# Autodesk Inventor assembly: Assembly1
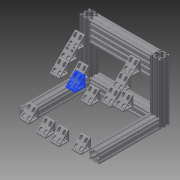
[picture p0: Inventor's stored thumbnail of the model, 180x180]
Saved by Autodesk Inventor 2014 (Build 180170000, 170)
## iProperties
Created: 2014-08-08
Part Number: Assembly1
Document SubType Name: Assembly
Designer: Matthew
Author: Matthew
## Documents named in this file (4)
- C:\Users\Matthew\Documents\GitHub\CNC Mill\Imported Components\8020-2020\Assembly1.iam
- C:\Users\Matthew\Documents\GitHub\CNC Mill\Imported Components\8020-2020\Part2.ipt
- C:\Users\Matthew\Documents\GitHub\CNC Mill\Imported Components\8020-2040\Assembly2.iam
- C:\Users\Matthew\Documents\GitHub\CNC Mill\Imported Components\8020-DEFAULT\Assembly3.iam
## Components (20 placed, 3 different names)
1. Part2:1 — Mate:5, Flush:3, Flush:4, Mate:7, Flush:7, Flush:8
2. Part2:2 — Flush:1, Flush:2, Mate:1, Mate:3, Mate:4
3. Part2:3 — Flush:1, Flush:2, Mate:1, Mate:2, Mate:5, Flush:3, Flush:4, Mate:6, Flush:5, Flush:6
4. Assembly2:1 [sub-assembly] — Mate:6, Flush:5, Flush:6
5. Assembly3:1 [sub-assembly] — Mate:2, Mate:3, Mate:4
6. Part2:4 — Mate:7, Flush:7, Flush:8, Mate:8, Flush:9, Flush:10
7. Part2:5 — Mate:8, Flush:9, Flush:10
8. Assembly3:2 [sub-assembly]
9. Assembly3:3 [sub-assembly]
10. Assembly3:4 [sub-assembly]
11. Assembly3:5 [sub-assembly]
12. Assembly3:6 [sub-assembly]
13. Assembly3:7 [sub-assembly]
14. Assembly3:8 [sub-assembly]
15. Assembly3:9 [sub-assembly]
16. Assembly3:10 [sub-assembly]
17. Assembly3:11 [sub-assembly]
18. Assembly3:12 [sub-assembly]
19. Assembly3:13 [sub-assembly]
20. Assembly3:14 [sub-assembly]
## Relationships (18: Flush 10, Mate 8)
- Flush:1: Part2:2 ↔ Part2:3
- Flush:2: Part2:2 ↔ Part2:3
- Mate:1: Part2:2 ↔ Part2:3
- Mate:2: Part2:3 ↔ Assembly3:1
- Mate:3: Part2:2 ↔ Assembly3:1
- Mate:4: Part2:2 ↔ Assembly3:1
- Mate:5: Part2:1 ↔ Part2:3
- Flush:3: Part2:1 ↔ Part2:3
- Flush:4: Part2:1 ↔ Part2:3
- Mate:6: Part2:3 ↔ Assembly2:1
- Flush:5: Part2:3 ↔ Assembly2:1
- Flush:6: Part2:3 ↔ Assembly2:1
- Mate:7: Part2:1 ↔ Part2:4
- Flush:7: Part2:1 ↔ Part2:4
- Flush:8: Part2:1 ↔ Part2:4
- Mate:8: Part2:4 ↔ Part2:5
- Flush:9: Part2:4 ↔ Part2:5
- Flush:10: Part2:4 ↔ Part2:5
